# Autodesk Inventor assembly: climber_assembly
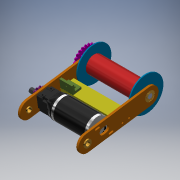
[picture p0: Inventor's stored thumbnail of the model, 180x180]
Saved by Autodesk Inventor 2017 (Build 210142000, 142)
## iProperties
Created: 2017-01-26
Part Number: climber_assembly
Document SubType Name: Assembly
Designer: Ben
Author: Ben
Revision Number: ANY
## Documents named in this file (13)
- C:\Users\Ben\Desktop\Projects\2017 Robot\Winch\climber_assembly.iam
- C:\Users\Ben\Desktop\Projects\2017 Robot\Winch\v2-VersaPlanetary-1stage-with-CIM.iam
- C:\Users\Ben\Desktop\Projects\2017 Robot\Winch\climber_cross_piece.ipt
- C:\Users\Ben\Desktop\Projects\2017 Robot\Winch\217-3875-STEP-20140818.ipt
- C:\Users\Ben\Desktop\Projects\2017 Robot\Winch\lift_drum_shield.ipt
- C:\Users\Ben\Desktop\Projects\2017 Robot\Winch\lift_drum_shaft.ipt
- C:\Users\Ben\Desktop\Projects\2017 Robot\Winch\217-2662-STEP-20140807.ipt
- C:\Users\Ben\Desktop\Projects\2017 Robot\Winch\217-2592-STEP-20140805.ipt
- C:\Users\Ben\Desktop\Projects\2017 Robot\Winch\217-2655.20121204.ipt
- C:\Users\Ben\Desktop\Projects\2017 Robot\Winch\Tension Angle.ipt
- C:\Users\Ben\Desktop\Projects\2017 Robot\Winch\6338K418_OIL-EMBEDDED FLANGED SLEEVE BRNG_6338K418.ipt
- C:\Users\Ben\Desktop\Projects\2017 Robot\Winch\Arm Plates.ipt
- C:\Users\Ben\Desktop\Projects\2017 Robot\Winch\winch drum.ipt
## Components (16 placed, 14 different names)
1. v2-VersaPlanetary-1stage-with-CIM_9 [sub-assembly] — Mate:7, Insert:14, Angle:2
2. climber_cross_piece_10 — Mate:9, Flush:2, Insert:12, Angle:1
3. 217-3875-STEP-20140818_12 — Insert:10, Insert:13
4. 217-3875-STEP-20140818_13 — Mate:1, Mate:2, Insert:7, Flush:1, Insert:11
5. lift_drum_shield_15 — Insert:13, Insert:15
6. lift_drum_shield_16 — Insert:7, Insert:16
7. lift_drum_shaft_17 — Mate:1, Mate:2, Flush:1, Mate:10, Mate:11, Flush:3
8. 217-2662-STEP-20140807_18 — Mate:7
9. 217-2592-STEP-20140805_19 — Mate:3, Mate:4, Mate:10, Mate:11, Flush:3
10. 217-2655.20121204_20 — Mate:3, Mate:4
11. Tension Angle:1 — Mate:9, Flush:2, Mate:12
12. 6338K418_OIL-EMBEDDED FLANGED SLEEVE BRNG_6338K418:1 — Insert:9
13. 6338K418_OIL-EMBEDDED FLANGED SLEEVE BRNG_6338K418:2 — Insert:8
14. Arm Plates:1 — Insert:8, Insert:10, Mate:12, Symmetry:1, Insert:14, Angle:2, Flush:4
15. Arm Plates:2 — Insert:9, Insert:11, Insert:12, Angle:1, Symmetry:1, Flush:4
16. winch drum:1 — Insert:15, Insert:16
## Relationships (26: Insert 10, Mate 9, Flush 4, Angle 2, Symmetry 1)
- Mate:1: 217-3875-STEP-20140818_13 ↔ lift_drum_shaft_17
- Mate:2: 217-3875-STEP-20140818_13 ↔ lift_drum_shaft_17
- Insert:7 (3.175 mm): 217-3875-STEP-20140818_13 ↔ lift_drum_shield_16
- Mate:3: 217-2592-STEP-20140805_19 ↔ 217-2655.20121204_20
- Mate:4: 217-2592-STEP-20140805_19 ↔ 217-2655.20121204_20
- Flush:1: 217-3875-STEP-20140818_13 ↔ lift_drum_shaft_17
- Mate:7: v2-VersaPlanetary-1stage-with-CIM_9 ↔ 217-2662-STEP-20140807_18
- Mate:9: climber_cross_piece_10 ↔ Tension Angle:1
- Flush:2: climber_cross_piece_10 ↔ Tension Angle:1
- Insert:8: 6338K418_OIL-EMBEDDED FLANGED SLEEVE BRNG_6338K418:2 ↔ Arm Plates:1
- Insert:9: 6338K418_OIL-EMBEDDED FLANGED SLEEVE BRNG_6338K418:1 ↔ Arm Plates:2
- Insert:10: 217-3875-STEP-20140818_12 ↔ Arm Plates:1
- Insert:11: 217-3875-STEP-20140818_13 ↔ Arm Plates:2
- Insert:12: climber_cross_piece_10 ↔ Arm Plates:2
- Angle:1 (0 deg): climber_cross_piece_10 ↔ Arm Plates:2
- Mate:10: lift_drum_shaft_17 ↔ 217-2592-STEP-20140805_19
- Mate:11: lift_drum_shaft_17 ↔ 217-2592-STEP-20140805_19
- Insert:13 (3.175 mm): 217-3875-STEP-20140818_12 ↔ lift_drum_shield_15
- Flush:3: lift_drum_shaft_17 ↔ 217-2592-STEP-20140805_19
- Mate:12: Tension Angle:1 ↔ Arm Plates:1
- Symmetry:1: Arm Plates:1 ↔ Arm Plates:2
- Insert:14: v2-VersaPlanetary-1stage-with-CIM_9 ↔ Arm Plates:1
- Angle:2 (0 deg): v2-VersaPlanetary-1stage-with-CIM_9 ↔ Arm Plates:1
- Flush:4: Arm Plates:1 ↔ Arm Plates:2
- Insert:15: lift_drum_shield_15 ↔ winch drum:1
- Insert:16: lift_drum_shield_16 ↔ winch drum:1
